# Autodesk Inventor assembly: Base
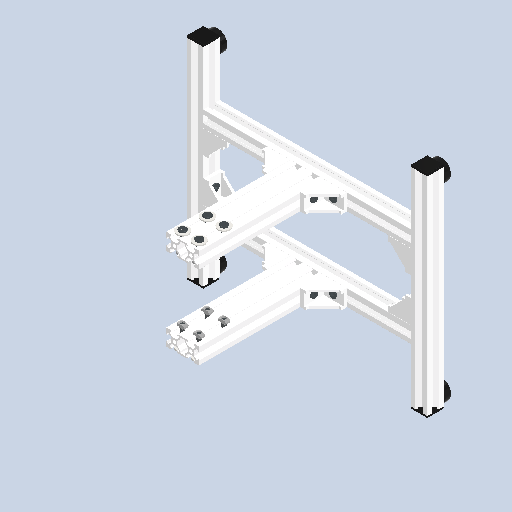
[picture p0: Inventor's stored thumbnail of the model, 512x512]
Saved by Autodesk Inventor 2022 (Build 260153000, 153)
## iProperties
Created: 2021-11-09
Part Number: Base
Document SubType Name: Assembly
Designer: JK
Author: JK
## Documents named in this file (6)
- C:\Users\JK\Documents\Inventor\UTM\Base.iam
- C:\Users\JK\Documents\Inventor\UTM\Vslot20x20x250mm.ipt
- C:\Users\JK\Documents\Inventor\UTM\ConjuntoUnion90GradosPerfil2020.iam
- C:\Users\JK\Documents\Inventor\UTM\Tapa plastica perfil 2020 Cimech 3D.ipt
- C:\Users\JK\Documents\Inventor\UTM\RubberFootAssembly.iam
- C:\Users\JK\Documents\Inventor\UTM\AluminiumProfileAssembly.iam
## Components (22 placed, 5 different names)
1. Vslot20x20x250mm:1 — Nivelación:28, Coincidencia:27
2. Vslot20x20x250mm:2 — Coincidencia:27
3. Vslot20x20x250mm:3
4. Vslot20x20x250mm:4 — Nivelación:29, Nivelación:30, Coincidencia:28, Nivelación:32, Coincidencia:29
5. ConjuntoUnion90GradosPerfil2020:1 [sub-assembly]
6. ConjuntoUnion90GradosPerfil2020:2 [sub-assembly]
7. ConjuntoUnion90GradosPerfil2020:3 [sub-assembly]
8. ConjuntoUnion90GradosPerfil2020:4 [sub-assembly]
9. Tapa plastica perfil 2020 Cimech 3D:1
10. Tapa plastica perfil 2020 Cimech 3D:2
11. Tapa plastica perfil 2020 Cimech 3D:3
12. ConjuntoUnion90GradosPerfil2020:5 [sub-assembly]
13. ConjuntoUnion90GradosPerfil2020:6 [sub-assembly] — Nivelación:28, Coincidencia:26
14. ConjuntoUnion90GradosPerfil2020:7 [sub-assembly]
15. ConjuntoUnion90GradosPerfil2020:8 [sub-assembly]
16. RubberFootAssembly:1 [sub-assembly]
17. RubberFootAssembly:2 [sub-assembly]
18. RubberFootAssembly:3 [sub-assembly]
19. AluminiumProfileAssembly:1 [sub-assembly] — Nivelación:27
20. AluminiumProfileAssembly:2 [sub-assembly] — Nivelación:27, Coincidencia:26
21. Tapa plastica perfil 2020 Cimech 3D:4 — Nivelación:29, Nivelación:30, Coincidencia:28, Nivelación:31
22. RubberFootAssembly:4 [sub-assembly] — Nivelación:31, Nivelación:32, Coincidencia:29
## Relationships (61: Flush 32, Mate 29)
- [Mate]: Vslot20x20x250mm:2 ↔ AluminiumProfileAssembly:1
- [Mate]: Vslot20x20x250mm:1 ↔ Vslot20x20x250mm:3
- [Flush]: Vslot20x20x250mm:2 ↔ Vslot20x20x250mm:3
- [Mate]: Vslot20x20x250mm:2 ↔ Vslot20x20x250mm:3
- [Mate]: Vslot20x20x250mm:1 ↔ Vslot20x20x250mm:4
- [Flush]: Vslot20x20x250mm:3 ↔ Vslot20x20x250mm:4
- [Flush]: Vslot20x20x250mm:2 ↔ Vslot20x20x250mm:4
- [Flush]: Vslot20x20x250mm:2 ↔ AluminiumProfileAssembly:1
- [Flush] (-65 mm): Vslot20x20x250mm:3 ↔ AluminiumProfileAssembly:1
- [Mate]: Vslot20x20x250mm:3 ↔ ConjuntoUnion90GradosPerfil2020:3
- [Flush]: Vslot20x20x250mm:3 ↔ ConjuntoUnion90GradosPerfil2020:3
- [Mate]: Vslot20x20x250mm:2 ↔ ConjuntoUnion90GradosPerfil2020:3
- [Mate]: Vslot20x20x250mm:3 ↔ ConjuntoUnion90GradosPerfil2020:1
- [Mate]: Vslot20x20x250mm:1 ↔ ConjuntoUnion90GradosPerfil2020:1
- [Flush]: Vslot20x20x250mm:3 ↔ ConjuntoUnion90GradosPerfil2020:1
- [Mate]: Vslot20x20x250mm:1 ↔ ConjuntoUnion90GradosPerfil2020:2
- [Mate]: Vslot20x20x250mm:2 ↔ ConjuntoUnion90GradosPerfil2020:4
- [Flush]: ConjuntoUnion90GradosPerfil2020:2 ↔ ConjuntoUnion90GradosPerfil2020:4
- [Flush]: ConjuntoUnion90GradosPerfil2020:1 ↔ ConjuntoUnion90GradosPerfil2020:2
- [Mate]: Vslot20x20x250mm:4 ↔ ConjuntoUnion90GradosPerfil2020:2
- [Mate]: Vslot20x20x250mm:4 ↔ ConjuntoUnion90GradosPerfil2020:4
- [Flush]: Vslot20x20x250mm:3 ↔ Tapa plastica perfil 2020 Cimech 3D:2
- [Flush]: Vslot20x20x250mm:3 ↔ Tapa plastica perfil 2020 Cimech 3D:1
- [Flush]: Vslot20x20x250mm:4 ↔ Tapa plastica perfil 2020 Cimech 3D:3
- [Flush]: Vslot20x20x250mm:3 ↔ Tapa plastica perfil 2020 Cimech 3D:2
- [Flush]: Vslot20x20x250mm:4 ↔ Tapa plastica perfil 2020 Cimech 3D:3
- [Flush]: Vslot20x20x250mm:3 ↔ Tapa plastica perfil 2020 Cimech 3D:1
- [Mate]: Vslot20x20x250mm:3 ↔ Tapa plastica perfil 2020 Cimech 3D:2
- [Mate]: Vslot20x20x250mm:4 ↔ Tapa plastica perfil 2020 Cimech 3D:3
- [Mate]: Vslot20x20x250mm:3 ↔ Tapa plastica perfil 2020 Cimech 3D:1
- [Mate]: Vslot20x20x250mm:2 ↔ ConjuntoUnion90GradosPerfil2020:5
- [Mate]: Vslot20x20x250mm:1 ↔ ConjuntoUnion90GradosPerfil2020:6
- [Mate]: Vslot20x20x250mm:1 ↔ ConjuntoUnion90GradosPerfil2020:7
- [Mate]: Vslot20x20x250mm:2 ↔ ConjuntoUnion90GradosPerfil2020:8
- [Flush]: ConjuntoUnion90GradosPerfil2020:5 ↔ AluminiumProfileAssembly:1
- [Flush]: ConjuntoUnion90GradosPerfil2020:8 ↔ AluminiumProfileAssembly:1
- [Mate]: ConjuntoUnion90GradosPerfil2020:8 ↔ AluminiumProfileAssembly:1
- [Mate]: ConjuntoUnion90GradosPerfil2020:5 ↔ AluminiumProfileAssembly:1
- [Mate]: Vslot20x20x250mm:3 ↔ RubberFootAssembly:3
- [Mate]: Vslot20x20x250mm:4 ↔ RubberFootAssembly:2
- [Mate]: Vslot20x20x250mm:3 ↔ RubberFootAssembly:1
- [Flush] (10 mm): Tapa plastica perfil 2020 Cimech 3D:2 ↔ RubberFootAssembly:3
- [Flush] (4.5 mm): Vslot20x20x250mm:3 ↔ RubberFootAssembly:3
- [Flush] (10 mm): Tapa plastica perfil 2020 Cimech 3D:1 ↔ RubberFootAssembly:1
- [Flush] (4.5 mm): Vslot20x20x250mm:3 ↔ RubberFootAssembly:1
- [Flush] (10 mm): Tapa plastica perfil 2020 Cimech 3D:3 ↔ RubberFootAssembly:2
- [Flush] (4.5 mm): Vslot20x20x250mm:4 ↔ RubberFootAssembly:2
- [Flush]: Vslot20x20x250mm:1 ↔ Vslot20x20x250mm:3
- [Mate]: Vslot20x20x250mm:1 ↔ AluminiumProfileAssembly:2
- [Flush]: Vslot20x20x250mm:1 ↔ AluminiumProfileAssembly:2
- [Flush] (125 mm): Vslot20x20x250mm:3 ↔ AluminiumProfileAssembly:2
- Nivelación:27 [Flush]: AluminiumProfileAssembly:1 ↔ AluminiumProfileAssembly:2
- Nivelación:28 [Flush]: Vslot20x20x250mm:1 ↔ ConjuntoUnion90GradosPerfil2020:6
- Coincidencia:26 [Mate]: ConjuntoUnion90GradosPerfil2020:6 ↔ AluminiumProfileAssembly:2
- Coincidencia:27 [Mate] (80 mm): Vslot20x20x250mm:1 ↔ Vslot20x20x250mm:2
- Nivelación:29 [Flush]: Vslot20x20x250mm:4 ↔ Tapa plastica perfil 2020 Cimech 3D:4
- Nivelación:30 [Flush]: Vslot20x20x250mm:4 ↔ Tapa plastica perfil 2020 Cimech 3D:4
- Coincidencia:28 [Mate]: Vslot20x20x250mm:4 ↔ Tapa plastica perfil 2020 Cimech 3D:4
- Nivelación:31 [Flush] (10 mm): Tapa plastica perfil 2020 Cimech 3D:4 ↔ RubberFootAssembly:4
- Nivelación:32 [Flush] (4.5 mm): Vslot20x20x250mm:4 ↔ RubberFootAssembly:4
- Coincidencia:29 [Mate]: Vslot20x20x250mm:4 ↔ RubberFootAssembly:4
